# Autodesk Inventor assembly: Overall_Assembly_Rev1
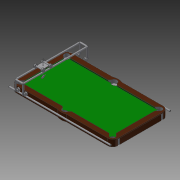
[picture p0: Inventor's stored thumbnail of the model, 180x180]
Saved by Autodesk Inventor 2015 (Build 190159000, 159)
## iProperties
Created: 2016-12-21
Part Number: Overall_Assembly_Rev1
Document SubType Name: Assembly
Designer: Guy
Author: Guy
## Documents named in this file (8)
- C:\Users\Guy\Documents\Fourth Year\Capstone\git\Capstone-Project\doc\CAD\LowLevel_Rev1\Overall_Assembly_Rev1.iam
- C:\Users\Guy\Documents\Fourth Year\Capstone\git\Capstone-Project\doc\CAD\Pool Table\Table_Model.ipt
- C:\Users\Guy\Documents\Fourth Year\Capstone\git\Capstone-Project\doc\CAD\LowLevel_Rev1\X_Rail-Rod-Rev1.ipt
- C:\Users\Guy\Documents\Fourth Year\Capstone\git\Capstone-Project\doc\CAD\LowLevel_Rev1\XY_Wheel-Rod-Rev1.ipt
- C:\Users\Guy\Documents\Fourth Year\Capstone\git\Capstone-Project\doc\CAD\LowLevel_Rev1\Y_Rail_Bridge-Rod-Rev1.ipt
- C:\Users\Guy\Documents\Fourth Year\Capstone\git\Capstone-Project\doc\CAD\LowLevel_Rev1\EE_Base-Rod-Rev1.ipt
- C:\Users\Guy\Documents\Fourth Year\Capstone\git\Capstone-Project\doc\CAD\LowLevel_Rev1\EE_Arm-Rod-Rev1.ipt
- C:\Users\Guy\Documents\Fourth Year\Capstone\git\Capstone-Project\doc\CAD\LowLevel_Rev1\EE-Rod-Rev1.ipt
## Components (15 placed, 7 different names)
1. Table_Model:1 — Flush:3, Tangent:1, Tangent:2, Angle:1, Tangent:3, Mate:32
2. X_Rail-Rod-Rev1:1 — Flush:3, Tangent:1, Tangent:2, Angle:1, Mate:2, Mate:3, Mate:4, Mate:5, Angle:2, Angle:3, Mate:7, Flush:4
3. X_Rail-Rod-Rev1:2 — Tangent:3, Angle:2, Angle:3, Mate:7, Flush:4, Mate:8, Mate:9, Mate:10, Mate:11
4. XY_Wheel-Rod-Rev1:1 — Mate:2, Mate:3, Mate:6, Mate:13, Mate:16
5. XY_Wheel-Rod-Rev1:2 — Mate:4, Mate:5, Mate:6, Mate:12, Mate:14, Mate:15
6. XY_Wheel-Rod-Rev1:3 — Mate:8, Mate:9, Mate:13
7. XY_Wheel-Rod-Rev1:4 — Mate:10, Mate:11, Mate:12
8. Y_Rail_Bridge-Rod-Rev1:1 — Mate:14, Mate:15, Mate:16, Angle:4, Mate:17, Mate:18, Mate:19, Mate:20, Mate:21, Mate:22, Mate:24, Mate:25
9. XY_Wheel-Rod-Rev1:1 — Mate:17, Mate:25, Mate:26, Mate:27
10. XY_Wheel-Rod-Rev1:2 — Mate:18, Mate:24, Mate:26, Mate:28
11. XY_Wheel-Rod-Rev1:3 — Mate:19, Mate:22, Mate:23, Mate:27, Mate:30
12. XY_Wheel-Rod-Rev1:4 — Mate:20, Mate:21, Mate:23, Mate:29
13. EE_Base-Rod-Rev1:1 — Mate:28, Mate:29, Mate:30, Mate:31, Mate:35
14. EE_Arm-Rod-Rev1:1 — Mate:31, Mate:32, Mate:33, Flush:5, Mate:34, Mate:35, Mate:36
15. EE-Rod-Rev1:1 — Mate:33, Flush:5, Mate:34, Mate:36
## Relationships (45: Mate 35, Angle 4, Flush 3, Tangent 3)
- Flush:3: Table_Model:1 ↔ X_Rail-Rod-Rev1:1
- Tangent:1 (24.6 mm): Table_Model:1 ↔ X_Rail-Rod-Rev1:1
- Tangent:2 (-70 mm): Table_Model:1 ↔ X_Rail-Rod-Rev1:1
- Angle:1 (0 deg): Table_Model:1 ↔ X_Rail-Rod-Rev1:1
- Mate:2: X_Rail-Rod-Rev1:1 ↔ XY_Wheel-Rod-Rev1:1
- Mate:3 (-40 mm): X_Rail-Rod-Rev1:1 ↔ XY_Wheel-Rod-Rev1:1
- Mate:4: X_Rail-Rod-Rev1:1 ↔ XY_Wheel-Rod-Rev1:2
- Mate:5 (-40 mm): X_Rail-Rod-Rev1:1 ↔ XY_Wheel-Rod-Rev1:2
- Mate:6 (150 mm): XY_Wheel-Rod-Rev1:1 ↔ XY_Wheel-Rod-Rev1:2
- Tangent:3 (24.6 mm): Table_Model:1 ↔ X_Rail-Rod-Rev1:2
- Angle:2 (0 deg): X_Rail-Rod-Rev1:1 ↔ X_Rail-Rod-Rev1:2
- Angle:3 (0 deg): X_Rail-Rod-Rev1:1 ↔ X_Rail-Rod-Rev1:2
- Mate:7: X_Rail-Rod-Rev1:1 ↔ X_Rail-Rod-Rev1:2
- Flush:4: X_Rail-Rod-Rev1:1 ↔ X_Rail-Rod-Rev1:2
- Mate:8: X_Rail-Rod-Rev1:2 ↔ XY_Wheel-Rod-Rev1:3
- Mate:9 (-40 mm): X_Rail-Rod-Rev1:2 ↔ XY_Wheel-Rod-Rev1:3
- Mate:10: X_Rail-Rod-Rev1:2 ↔ XY_Wheel-Rod-Rev1:4
- Mate:11 (-40 mm): X_Rail-Rod-Rev1:2 ↔ XY_Wheel-Rod-Rev1:4
- Mate:12: XY_Wheel-Rod-Rev1:2 ↔ XY_Wheel-Rod-Rev1:4
- Mate:13: XY_Wheel-Rod-Rev1:1 ↔ XY_Wheel-Rod-Rev1:3
- Mate:14: XY_Wheel-Rod-Rev1:2 ↔ Y_Rail_Bridge-Rod-Rev1:1
- Mate:15: XY_Wheel-Rod-Rev1:2 ↔ Y_Rail_Bridge-Rod-Rev1:1
- Mate:16: XY_Wheel-Rod-Rev1:1 ↔ Y_Rail_Bridge-Rod-Rev1:1
- Angle:4 (-180 deg): Y_Rail_Bridge-Rod-Rev1:1
- Mate:17: Y_Rail_Bridge-Rod-Rev1:1 ↔ XY_Wheel-Rod-Rev1:1
- Mate:18: Y_Rail_Bridge-Rod-Rev1:1 ↔ XY_Wheel-Rod-Rev1:2
- Mate:19 (150 mm): Y_Rail_Bridge-Rod-Rev1:1 ↔ XY_Wheel-Rod-Rev1:3
- Mate:20 (150 mm): Y_Rail_Bridge-Rod-Rev1:1 ↔ XY_Wheel-Rod-Rev1:4
- Mate:21 (-40 mm): Y_Rail_Bridge-Rod-Rev1:1 ↔ XY_Wheel-Rod-Rev1:4
- Mate:22 (-40 mm): Y_Rail_Bridge-Rod-Rev1:1 ↔ XY_Wheel-Rod-Rev1:3
- Mate:23 (150 mm): XY_Wheel-Rod-Rev1:3 ↔ XY_Wheel-Rod-Rev1:4
- Mate:24 (-40 mm): Y_Rail_Bridge-Rod-Rev1:1 ↔ XY_Wheel-Rod-Rev1:2
- Mate:25 (-40 mm): Y_Rail_Bridge-Rod-Rev1:1 ↔ XY_Wheel-Rod-Rev1:1
- Mate:26 (150 mm): XY_Wheel-Rod-Rev1:1 ↔ XY_Wheel-Rod-Rev1:2
- Mate:27: XY_Wheel-Rod-Rev1:1 ↔ XY_Wheel-Rod-Rev1:3
- Mate:28: XY_Wheel-Rod-Rev1:2 ↔ EE_Base-Rod-Rev1:1
- Mate:29: XY_Wheel-Rod-Rev1:4 ↔ EE_Base-Rod-Rev1:1
- Mate:30: XY_Wheel-Rod-Rev1:3 ↔ EE_Base-Rod-Rev1:1
- Mate:31: EE_Base-Rod-Rev1:1 ↔ EE_Arm-Rod-Rev1:1
- Mate:32 (100 mm): Table_Model:1 ↔ EE_Arm-Rod-Rev1:1
- Mate:33: EE_Arm-Rod-Rev1:1 ↔ EE-Rod-Rev1:1
- Flush:5 (5 mm): EE_Arm-Rod-Rev1:1 ↔ EE-Rod-Rev1:1
- Mate:34 (40 mm): EE_Arm-Rod-Rev1:1 ↔ EE-Rod-Rev1:1
- Mate:35 (100 mm): EE_Base-Rod-Rev1:1 ↔ EE_Arm-Rod-Rev1:1
- Mate:36 (40 mm): EE_Arm-Rod-Rev1:1 ↔ EE-Rod-Rev1:1
